# Autodesk Inventor assembly: ASY Мешалка
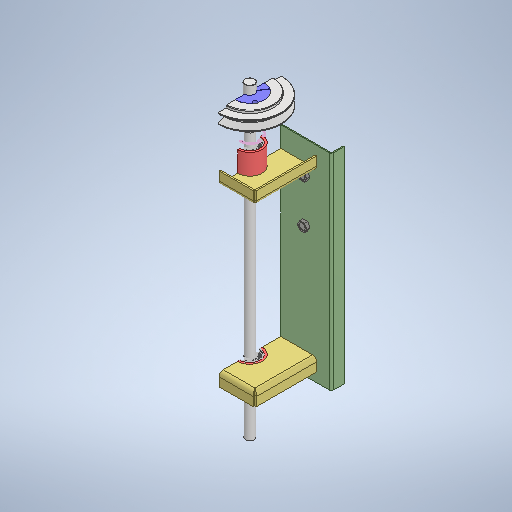
[picture p0: Inventor's stored thumbnail of the model, 512x512]
Saved by Autodesk Inventor 2025 (Build 290162010, 162A)
## iProperties
Created: 2024-04-09
Part Number: ASY Мешалка
Document SubType Name: Assembly
Designer: pokla
Stock Number: ASY Мешалка
Author: pokla
## Documents named in this file (14)
- C:\Users\admin\YandexDisk-badmisterfox\домашниий пк\Inventor\tale tales\Gusev_Meshalka\ASY Мешалка\ASY Мешалка.iam
- C:\Users\admin\YandexDisk-badmisterfox\домашниий пк\Inventor\tale tales\Gusev_Meshalka\ASY Мешалка\SKF B7203 BE.ipt
- C:\Users\admin\YandexDisk-badmisterfox\домашниий пк\Inventor\tale tales\Gusev_Meshalka\ASY Мешалка\CSN 02 9401 - G 17x40x7 - NBR.ipt
- C:\Users\admin\YandexDisk-badmisterfox\домашниий пк\Inventor\tale tales\Gusev_Meshalka\ASY Мешалка\Шкив 119 мм.ipt
- Шкив 119 мм.ipt
- C:\Users\admin\YandexDisk-badmisterfox\домашниий пк\Inventor\tale tales\Gusev_Meshalka\ASY Мешалка\Втулка для шкива.ipt
- C:\Users\admin\YandexDisk-badmisterfox\домашниий пк\Inventor\tale tales\Gusev_Meshalka\ASY Мешалка\ANSI B 27.7M - 3AMI-17.ipt
- C:\Users\admin\YandexDisk-badmisterfox\домашниий пк\Inventor\tale tales\Gusev_Meshalka\ASY Мешалка\ANSI B 27.7M - 3BMI-40.ipt
- C:\Users\admin\YandexDisk-badmisterfox\домашниий пк\Inventor\tale tales\Gusev_Meshalka\ASY Мешалка\Корпус.iam
- C:\Users\admin\YandexDisk-badmisterfox\домашниий пк\Inventor\tale tales\Gusev_Meshalka\ASY Мешалка\Седло для сальника.ipt
- C:\Users\admin\YandexDisk-badmisterfox\домашниий пк\Inventor\tale tales\Gusev_Meshalka\ASY Мешалка\Седло для подшипника.ipt
- C:\Users\admin\YandexDisk-badmisterfox\домашниий пк\Inventor\tale tales\Gusev_Meshalka\ASY Мешалка\Shaft1.ipt
- C:\Users\admin\YandexDisk-badmisterfox\домашниий пк\Inventor\tale tales\Gusev_Meshalka\ASY Мешалка\Кожух.ipt
- C:\Users\admin\YandexDisk-badmisterfox\домашниий пк\Inventor\tale tales\Gusev_Meshalka\ASY Мешалка\Крепление корпуса.ipt
## Components (19 placed, 16 different names)
1. SKF B7203 BE.ipt:1
2. SKF B7203 BE.ipt:2
3. CSN 02 9401 - G 17x40x7 - NBR.ipt:1
4. CSN 02 9401 - G 17x40x7 - NBR.ipt:2 — Mate:5
5. Шкив 119 мм.ipt:1 — Rigid:18
6. Втулка для шкива.ipt:1 — Rigid:18, Rigid:19
7. ANSI B 27.7M - 3AMI-17.ipt:1 — Rigid:15
8. ANSI B 27.7M - 3BMI-40.ipt:2
9. Кожух.ipt:1
10. Крепление корпуса.ipt:1 — Flush:5, Mate:3, Flush:6, Rigid:20
11. Корпус.iam:1 [sub-assembly] — Flush:1, Flush:2, Flush:3, Flush:4, Mate:1, Flush:5, Mate:3
12. Седло для сальника.ipt:1
13. Седло для подшипника.ipt:1 — Rigid:20, Mate:4
14. Shaft:1 — Rigid:15, Rigid:19, Mate:4, Mate:5, Mate:6
15. Крепление корпуса:2 — Flush:4, Mate:1, Mate:2, Rigid:21
16. Седло для подшипника:2 — Rigid:21
17. CSN 02 9401 G G 17x40x7 - NBR:3 — Mate:6
18. SKF B- Angular contact SKF B7203 BE:4
19. CSN 02 9401 G G 17x40x7 - NBR:4
## Relationships (17: Flush 6, Mate 6, WeldJoint 5)
- Flush:1: Корпус.iam:1
- Flush:2: Корпус.iam:1
- Flush:3: Корпус.iam:1
- Rigid:15 [WeldJoint]: ANSI B 27.7M - 3AMI-17.ipt:1 ↔ Shaft:1
- Rigid:18 [WeldJoint]: Шкив 119 мм.ipt:1 ↔ Втулка для шкива.ipt:1
- Rigid:19 [WeldJoint] (-16.3 mm): Втулка для шкива.ipt:1 ↔ Shaft:1
- Flush:4 (18 mm): Корпус.iam:1 ↔ Крепление корпуса:2
- Mate:1: Корпус.iam:1 ↔ Крепление корпуса:2
- Mate:2: Крепление корпуса:2
- Flush:5 (18 mm): Крепление корпуса.ipt:1 ↔ Корпус.iam:1
- Mate:3: Крепление корпуса.ipt:1 ↔ Корпус.iam:1
- Flush:6: Крепление корпуса.ipt:1
- Rigid:20 [WeldJoint]: Крепление корпуса.ipt:1 ↔ Седло для подшипника.ipt:1
- Rigid:21 [WeldJoint]: Крепление корпуса:2 ↔ Седло для подшипника:2
- Mate:4: Седло для подшипника.ipt:1 ↔ Shaft:1
- Mate:5: CSN 02 9401 - G 17x40x7 - NBR.ipt:2 ↔ Shaft:1
- Mate:6: Shaft:1 ↔ CSN 02 9401 G G 17x40x7 - NBR:3
